# Autodesk Inventor assembly: Ani_Ani
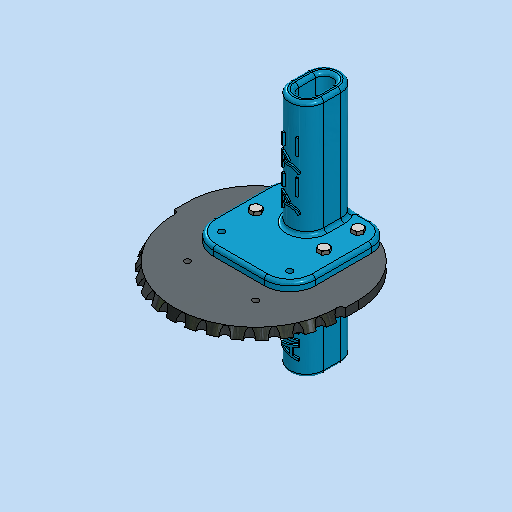
[picture p0: Inventor's stored thumbnail of the model, 512x512]
Saved by Autodesk Inventor 2026.1 (Build 301233000, 233)
## iProperties
Created: 2026-04-14
Part Number: Ani_Ani
Document SubType Name: Assembly
Designer: ADMIN
Author: ADMIN
## Documents named in this file (5)
- C:\Users\ADMIN\Documents\Documents\MECHATRONICS\5.2\Computer_Controlled_Manufacturing(Dr.Wamai)\Ani-Ani\Ani_Ani.iam
- C:\Users\ADMIN\Documents\Documents\MECHATRONICS\5.2\Computer_Controlled_Manufacturing(Dr.Wamai)\Ani-Ani\Blade.ipt
- C:\Users\ADMIN\Documents\Documents\MECHATRONICS\5.2\Computer_Controlled_Manufacturing(Dr.Wamai)\Ani-Ani\Handle.ipt
- C:\Users\ADMIN\Documents\Inventor\Content Center Files\R2026\en-US\CNS 3129\CNS 3129 - M 3 x 0.5.ipt
- C:\Users\ADMIN\Documents\Inventor\Content Center Files\R2026\en-US\BS 3692(3)\BS 3692 - M3 x 14(1).ipt
## Components (10 placed, 4 different names)
1. Blade:1 — Mate:1, Mate:2, Mate:3, Mate:17, Mate:18, Mate:19, Mate:20
2. Handle:1 — Mate:1, Mate:2, Mate:3, Mate:5, Mate:6, Mate:7, Mate:8, Mate:9, Mate:10, Mate:11, Mate:12
3. BS 3692 Hexagon Head Screw - Metric M3 x 14:1 — Mate:8, Mate:10, Mate:16
4. BS 3692 Hexagon Head Screw - Metric M3 x 14:2 — Mate:5, Mate:9, Mate:15
5. BS 3692 Hexagon Head Screw - Metric M3 x 14:3 — Mate:7, Mate:12, Mate:14
6. BS 3692 Hexagon Head Screw - Metric M3 x 14:4 — Mate:6, Mate:11, Mate:13
7. CNS 3129 M 3:1 — Mate:15, Mate:18
8. CNS 3129 M 3:2 — Mate:16, Mate:17
9. CNS 3129 M 3:3 — Mate:14, Mate:20
10. CNS 3129 M 3:4 — Mate:13, Mate:19
## Relationships (19: Mate 19)
- Mate:1: Blade:1 ↔ Handle:1
- Mate:2: Blade:1 ↔ Handle:1
- Mate:3: Blade:1 ↔ Handle:1
- Mate:5: Handle:1 ↔ BS 3692 Hexagon Head Screw - Metric M3 x 14:2
- Mate:6: Handle:1 ↔ BS 3692 Hexagon Head Screw - Metric M3 x 14:4
- Mate:7: Handle:1 ↔ BS 3692 Hexagon Head Screw - Metric M3 x 14:3
- Mate:8: Handle:1 ↔ BS 3692 Hexagon Head Screw - Metric M3 x 14:1
- Mate:9: Handle:1 ↔ BS 3692 Hexagon Head Screw - Metric M3 x 14:2
- Mate:10: Handle:1 ↔ BS 3692 Hexagon Head Screw - Metric M3 x 14:1
- Mate:11: Handle:1 ↔ BS 3692 Hexagon Head Screw - Metric M3 x 14:4
- Mate:12: Handle:1 ↔ BS 3692 Hexagon Head Screw - Metric M3 x 14:3
- Mate:13: BS 3692 Hexagon Head Screw - Metric M3 x 14:4 ↔ CNS 3129 M 3:4
- Mate:14: BS 3692 Hexagon Head Screw - Metric M3 x 14:3 ↔ CNS 3129 M 3:3
- Mate:15: BS 3692 Hexagon Head Screw - Metric M3 x 14:2 ↔ CNS 3129 M 3:1
- Mate:16: BS 3692 Hexagon Head Screw - Metric M3 x 14:1 ↔ CNS 3129 M 3:2
- Mate:17: Blade:1 ↔ CNS 3129 M 3:2
- Mate:18: Blade:1 ↔ CNS 3129 M 3:1
- Mate:19: Blade:1 ↔ CNS 3129 M 3:4
- Mate:20: Blade:1 ↔ CNS 3129 M 3:3
